# Autodesk Inventor assembly: Assembly
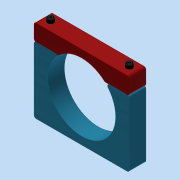
[picture p0: Inventor's stored thumbnail of the model, 180x180]
Saved by Autodesk Inventor 2017.3 (Build 213256000, 256)
## iProperties
Created: 2018-07-27
Part Number: Assembly
Document SubType Name: Assembly
Designer: Derek Wider
Author: Derek Wider
## Documents named in this file (5)
- G:\Projects\Submarine\Submarine-project\CAD\midships\HullFixturing\Assembly.iam
- G:\Projects\Submarine\Submarine-project\CAD\midships\HullFixturing\Bottom.ipt
- G:\Projects\Submarine\Submarine-project\CAD\midships\HullFixturing\Top.ipt
- G:\Projects\Submarine\Submarine-project\CAD\common\ThreadedRod_Nuts_Bolts\Bolt_SocketHead_Hex_Thread_.25_20_1.25.ipt
- G:\Projects\Submarine\Submarine-project\CAD\common\ThreadedRod_Nuts_Bolts\HexNutThread_.25_20.ipt
## Components (6 placed, 4 different names)
1. Bottom:1 — Mate:1, Mate:2, Flush:1, Mate:9, Mate:10, Angle:1, Angle:2
2. Top:1 — Mate:1, Mate:2, Flush:1, Mate:3, Mate:4, Mate:5, Mate:6
3. Bolt_SocketHead_Hex_Thread_.25_20_1.25:1 — Mate:4, Mate:6, Mate:8
4. Bolt_SocketHead_Hex_Thread_.25_20_1.25:2 — Mate:3, Mate:5, Mate:7
5. HexNutThread_.25_20:1 — Mate:8, Mate:10, Angle:2
6. HexNutThread_.25_20:2 — Mate:7, Mate:9, Angle:1
## Relationships (13: Mate 10, Angle 2, Flush 1)
- Mate:1: Bottom:1 ↔ Top:1
- Mate:2: Bottom:1 ↔ Top:1
- Flush:1: Bottom:1 ↔ Top:1
- Mate:3: Top:1 ↔ Bolt_SocketHead_Hex_Thread_.25_20_1.25:2
- Mate:4: Top:1 ↔ Bolt_SocketHead_Hex_Thread_.25_20_1.25:1
- Mate:5: Top:1 ↔ Bolt_SocketHead_Hex_Thread_.25_20_1.25:2
- Mate:6: Top:1 ↔ Bolt_SocketHead_Hex_Thread_.25_20_1.25:1
- Mate:7: Bolt_SocketHead_Hex_Thread_.25_20_1.25:2 ↔ HexNutThread_.25_20:2
- Mate:8: Bolt_SocketHead_Hex_Thread_.25_20_1.25:1 ↔ HexNutThread_.25_20:1
- Mate:9: Bottom:1 ↔ HexNutThread_.25_20:2
- Mate:10: Bottom:1 ↔ HexNutThread_.25_20:1
- Angle:1 (0 deg): Bottom:1 ↔ HexNutThread_.25_20:2
- Angle:2 (0 deg): Bottom:1 ↔ HexNutThread_.25_20:1
